# Autodesk Inventor assembly: Cupboard
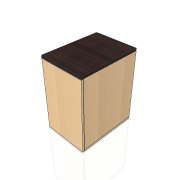
[picture p0: Inventor's stored thumbnail of the model, 180x180]
Saved by Autodesk Inventor 2024 (Build 280153000, 153)
## iProperties
RuleStatus: InUse
AfterAnyParamChange0: Configuration Control
AfterAnyUserParamChange0: Configuration Control
Created: 2023-03-29
Part Number: Cupboard
Document SubType Name: Assembly
Designer: sauliusd
Author: sauliusd
## Documents named in this file (10)
- C:\W4INV 2024 Design\PROJECTS\Samples\API Demo\iBox Insert\Cupboard.iam
- C:\W4INV 2024 Design\PROJECTS\Samples\API Demo\iBox Insert\Cupboard Left.ipt
- C:\W4INV 2024 Design\PROJECTS\Samples\API Demo\iBox Insert\Cupboard Top.ipt
- C:\W4INV 2024 Design\PROJECTS\Samples\API Demo\iBox Insert\Cupboard Bottom.ipt
- C:\W4INV 2024 Design\PROJECTS\Samples\API Demo\iBox Insert\Cupboard Right.ipt
- C:\W4INV 2024 Design\PROJECTS\Samples\API Demo\iBox Insert\Cupboard Back.ipt
- C:\W4INV 2024 Design\PROJECTS\Samples\API Demo\iBox Insert\Cupboard Shelf.ipt
- C:\W4INV 2024 Design\PROJECTS\Samples\API Demo\iBox Insert\Cupboard Door.ipt
- C:\W4INV 2024 Design\PROJECTS\Samples\API Demo\iBox Insert\Cupboard.ipt
- C:\W4INV 2024 Design\PROJECTS\Samples\API Demo\iBox Insert\Cupboard Drawers Facade.ipt
## Components (9 placed, 9 different names)
1. Skeleton — Flush:1, Flush:2, Flush:3
2. Cupboard Left
3. Cupboard Top
4. Cupboard Bottom
5. Cupboard Right
6. Cupboard Back
7. Cupboard Shelf
8. Cupboard Door
9. Cupboard Drawers Facade
## Relationships (3: Flush 3)
- Flush:1: Skeleton
- Flush:2: Skeleton
- Flush:3: Skeleton
